# Autodesk Inventor assembly: Supershifter Cluster Shaft subassembly
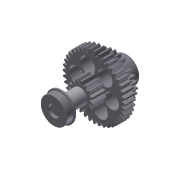
[picture p0: Inventor's stored thumbnail of the model, 180x180]
Saved by Autodesk Inventor 2011 (Build 150239000, 239)
## iProperties
Created: 2011-07-04
Part Number: Supershifter Cluster Shaft subassembly
Document SubType Name: Assembly
Designer: Dan Niemitalo
Mass: 199.079 g
Surface Area: 206.885 cm^2
Volume: 31.343 cm^3
Density: 6.35161 g/cm^3
Author: Dan Niemitalo
## Documents named in this file (8)
- H:\Nemo\Documents\Robotics\COTS Parts\Gearboxes\Shafts\Supershifter Cluster Shaft subassembly.iam
- H:\Nemo\Documents\Robotics\COTS Parts\Gearboxes\Spacers\Supershifter cluster spacer.ipt
- H:\Nemo\Documents\Robotics\COTS Parts\Gearboxes\Spacers\Washer - shifter spacing.ipt
- H:\Nemo\Documents\Robotics\COTS Parts\Gearboxes\Bearings\Bearing FR6zz.ipt
- H:\Nemo\Documents\Robotics\COTS Parts\Gearboxes\Shafts\Supershifter Cluster Shaft.ipt
- H:\Nemo\Documents\Robotics\COTS Parts\Gearboxes\Gears\Gear 20dp 375hex 15T.ipt
- H:\Nemo\Documents\Robotics\COTS Parts\Gearboxes\Gears\Gear 20dp 375hex 40T.ipt
- H:\Nemo\Documents\Robotics\COTS Parts\Gearboxes\Gears\Gear 20dp 375hex 28T.ipt
## Components (8 placed, 7 different names)
1. Washer - shifter spacing:1 — Mate:6, Mate:22
2. Bearing FR6zz:1
3. Bearing FR6zz:2
4. SS cluster shaft — Mate:2, Mate:6, Mate:16, Angle:4, Mate:18, Angle:5, Mate:20, Angle:6
5. SS cluster spacer — Mate:2
6. Gear 15T 20dp 375hex:1 — Mate:16, Angle:4, Mate:19
7. Gear 40T 20dp 375hex:1 — Mate:18, Angle:5, Mate:19, Mate:21
8. Gear 28T 20dp 375 hex:1 — Mate:20, Angle:6, Mate:21, Mate:22
## Relationships (17: Mate 14, Angle 3)
- [Mate]: Bearing FR6zz:1 ↔ SS cluster shaft
- Mate:2: SS cluster shaft ↔ SS cluster spacer
- Mate:6: Washer - shifter spacing:1 ↔ SS cluster shaft
- [Mate]: Bearing FR6zz:2 ↔ SS cluster shaft
- [Mate]: Washer - shifter spacing:1 ↔ Bearing FR6zz:2
- [Mate] (0.254 mm): Bearing FR6zz:1 ↔ SS cluster spacer
- [Mate] (-50.8 mm): Bearing FR6zz:1 ↔ Bearing FR6zz:2
- [Mate] (0.3429 mm): Bearing FR6zz:1 ↔ SS cluster shaft
- Mate:16: SS cluster shaft ↔ Gear 15T 20dp 375hex:1
- Angle:4 (0 deg): SS cluster shaft ↔ Gear 15T 20dp 375hex:1
- Mate:18: SS cluster shaft ↔ Gear 40T 20dp 375hex:1
- Angle:5 (0 deg): SS cluster shaft ↔ Gear 40T 20dp 375hex:1
- Mate:19: Gear 15T 20dp 375hex:1 ↔ Gear 40T 20dp 375hex:1
- Mate:20: SS cluster shaft ↔ Gear 28T 20dp 375 hex:1
- Angle:6 (0 deg): SS cluster shaft ↔ Gear 28T 20dp 375 hex:1
- Mate:21: Gear 40T 20dp 375hex:1 ↔ Gear 28T 20dp 375 hex:1
- Mate:22: Washer - shifter spacing:1 ↔ Gear 28T 20dp 375 hex:1
